# Autodesk Inventor assembly: M4-BallDevice
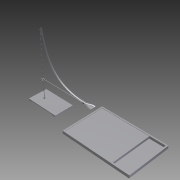
[picture p0: Inventor's stored thumbnail of the model, 180x180]
Saved by Autodesk Inventor 2012 SP2 (Build 160219200, 219)
## iProperties
Created: 2013-07-29
Part Number: M4-BallDevice
Document SubType Name: Assembly
Designer: 1
Author: 1
## Documents named in this file (3)
- D:\p3_metod1580library\figures\sources\M4-BallDevice\M4-BallDevice.iam
- D:\p3_metod1580library\figures\sources\M4-BallDevice\BallGuideAsmy.iam
- D:\p3_metod1580library\figures\sources\M4-BallDevice\CatcherBox.ipt
## Components (2 placed, 2 different names)
1. BallGuideAsmy:1 [sub-assembly] — Flush:1
2. CatcherBox:1 — Flush:5
## Relationships (4: Flush 4)
- Flush:1: BallGuideAsmy:1
- [Flush]: BallGuideAsmy:1
- [Flush]: BallGuideAsmy:1
- Flush:5: CatcherBox:1
